# Autodesk Inventor assembly: PistonTricep
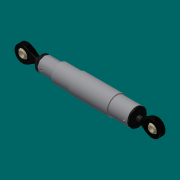
[picture p0: Inventor's stored thumbnail of the model, 180x180]
Saved by Autodesk Inventor 2015 SP1 (Build 190203100, 203)
## iProperties
Created: 2016-10-01
Part Number: PistonTricep
Document SubType Name: Assembly
Designer: Val
Author: Val
## Documents named in this file (6)
- C:\Users\Val\Desktop\ExoGit\elysium-max-exoskeleton\src\Assemblies\Pistons\PistonHipFront.iam
- C:\Users\Val\Desktop\ExoGit\elysium-max-exoskeleton\src\Pistons\PistonBodyCap.ipt
- C:\Users\Val\Desktop\ExoGit\elysium-max-exoskeleton\src\Pistons\PistonShaftCap.ipt
- C:\Users\Val\Desktop\ExoGit\elysium-max-exoskeleton\src\External\Bearing.iam
- C:\Users\Val\Desktop\ExoGit\elysium-max-exoskeleton\src\Pistons\PistonHipFrontShaft.ipt
- C:\Users\Val\Desktop\ExoGit\elysium-max-exoskeleton\src\Pistons\PistonHipFrontBody.ipt
## Components (6 placed, 5 different names)
1. PistonBodyCap:1 — Mate:3, Mate:4, Mate:7, Mate:8, Flush:1
2. PistonShaftCap:1 — Mate:5, Mate:6, Mate:11, Mate:12
3. PistonBody:1 — Mate:1, Mate:3, Mate:4, Mate:10, Mate:13
4. PistonShaft:1 — Mate:1, Mate:5, Mate:6, Mate:7, Angle:3
5. Bearing:1 [sub-assembly] — Mate:8, Angle:1, Flush:1
6. Bearing:2 [sub-assembly] — Mate:11, Mate:12, Angle:2
## Relationships (15: Mate 11, Angle 3, Flush 1)
- Mate:1: PistonBody:1 ↔ PistonShaft:1
- Mate:3: PistonBodyCap:1 ↔ PistonBody:1
- Mate:4: PistonBodyCap:1 ↔ PistonBody:1
- Mate:5: PistonShaftCap:1 ↔ PistonShaft:1
- Mate:6: PistonShaftCap:1 ↔ PistonShaft:1
- Mate:7 (10 mm): PistonBodyCap:1 ↔ PistonShaft:1
- Mate:8: PistonBodyCap:1 ↔ Bearing:1
- Angle:1 (0 deg): Bearing:1
- Mate:10: PistonBody:1
- Mate:11: PistonShaftCap:1 ↔ Bearing:2
- Mate:12 (5 mm): PistonShaftCap:1 ↔ Bearing:2
- Angle:2 (0 deg): Bearing:2
- Flush:1 (-10 mm): PistonBodyCap:1 ↔ Bearing:1
- Angle:3 (0 deg): PistonShaft:1
- Mate:13: PistonBody:1
